# Autodesk Inventor assembly: robot_driver_board
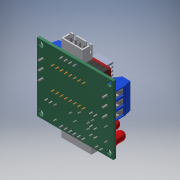
[picture p0: Inventor's stored thumbnail of the model, 180x180]
Saved by Autodesk Inventor 2019 (Build 230136000, 136)
## iProperties
Created: 2020-01-03
Part Number: robot_driver_board
Material: Типовые
Document SubType Name: Assembly
Designer: Петров Иван
Author: Петров Иван
## Documents named in this file (12)
- E:\IVAN\Ivan_desktop\GitHub\Arm_manip\electronic\3d_visualization\robot_driver_board\robot_driver_board.iam
- E:\IVAN\Ivan_desktop\GitHub\Arm_manip\electronic\3d_visualization\lib\tb5p-3p_p5_l15_w7-6_h10.ipt
- E:\IVAN\Ivan_desktop\GitHub\Arm_manip\electronic\3d_visualization\robot_driver_board\board.ipt
- E:\IVAN\Ivan_desktop\GitHub\Arm_manip\electronic\3d_visualization\lib\Female Pin Header 01x01 Pitch 2.54mm Height 8.5mm\Female Pin Header 01x01 Pitch 2.54mm Height 8.5mm.iam
- E:\IVAN\Ivan_desktop\GitHub\Arm_manip\electronic\3d_visualization\lib\A4988\A4988 RED.iam
- E:\IVAN\Ivan_desktop\GitHub\Arm_manip\electronic\3d_visualization\lib\LED 3mm (Red).ipt
- E:\IVAN\Ivan_desktop\GitHub\Arm_manip\electronic\3d_visualization\lib\JST - XH - Thru (R) - 4Pin - 2.54mm.ipt
- E:\IVAN\Ivan_desktop\GitHub\Arm_manip\electronic\3d_visualization\lib\JST - XH - Thru (R) - 6Pin - 2.54mm.ipt
- E:\IVAN\Ivan_desktop\GitHub\Arm_manip\electronic\3d_visualization\lib\JST - XH - Thru (V) - 4Pin - 2.54mm.ipt
- E:\IVAN\Ivan_desktop\GitHub\Arm_manip\electronic\3d_visualization\lib\JST - XH - Thru (V) - 6Pin - 2.54mm.ipt
- E:\IVAN\Ivan_desktop\GitHub\Arm_manip\electronic\3d_visualization\lib\1,2 kOhm R Axial DIN0207 L6.3mm D2.5mm P10.16mm Horizontal.ipt
- E:\IVAN\Ivan_desktop\GitHub\Arm_manip\electronic\3d_visualization\lib\1,0 kOhm R Axial DIN0207 L6.3mm D2.5mm P7.62mm Horizontal.ipt
## Components (34 placed, 11 different names)
1. tb5p-3p_p5_l15_w7-6_h10:1 — Совмещение:1, Совмещение:2, Совмещение:3
2. tb5p-3p_p5_l15_w7-6_h10:2 — Совмещение:4, Совмещение:5, Совмещение:6
3. board:1 — Совмещение:1, Совмещение:2, Совмещение:3, Совмещение:4, Совмещение:5, Совмещение:6, Совмещение:7, Совмещение:8, Угол:1, Совмещение:9, Совмещение:10, Угол:2, Совмещение:14, Совмещение:15, Совмещение:16, Совмещение:17, Совмещение:18, Совмещение:19, Совмещение:20, Совмещение:21, Совмещение:22, Совмещение:23, Совмещение:24, Совмещение:25, Совмещение:26, Совмещение:27, Совмещение:28, Совмещение:29, Совмещение:30, Совмещение:31, Совмещение:32, Совмещение:33, Совмещение:34, Совмещение:35, Совмещение:36, Совмещение:37, Совмещение:38, Совмещение:39, Совмещение:40, Совмещение:41, Совмещение:42, Касательность:1, Совмещение:43, Совмещение:44, Касательность:2, Касательность:3, Совмещение:45, Совмещение:46, Совмещение:47, Совмещение:48, Касательность:4, Совмещение:49, Совмещение:50, Касательность:5
4. A4988 RED:1 [sub-assembly] — Совмещение:11, Совмещение:12, Совмещение:13
5. LED 3mm (Red):1 — Совмещение:17, Совмещение:18, Совмещение:19
6. LED 3mm (Red):2 — Совмещение:14, Совмещение:15, Совмещение:16
7. LED 3mm (Red):3 — Совмещение:20, Совмещение:21, Совмещение:22
8. LED 3mm (Red):4 — Совмещение:23, Совмещение:24, Совмещение:25
9. LED 3mm (Red):5 — Совмещение:26, Совмещение:27, Совмещение:28
10. JST - XH - Thru (R) - 4Pin - 2.54mm:1 — Совмещение:29, Совмещение:30, Совмещение:31
11. JST - XH - Thru (R) - 6Pin - 2.54mm:1 — Совмещение:32, Совмещение:33, Совмещение:34
12. JST - XH - Thru (V) - 4Pin - 2.54mm:1 — Совмещение:35, Совмещение:36, Совмещение:37
13. JST - XH - Thru (V) - 6Pin - 2.54mm:1 — Совмещение:38, Совмещение:39, Совмещение:40
14. 1,2 kOhm R Axial DIN0207 L6.3mm D2.5mm P10.16mm Horizontal:1 — Совмещение:41, Совмещение:42, Касательность:1
15. 1,0 kOhm R Axial DIN0207 L6.3mm D2.5mm P7.62mm Horizontal:1 — Совмещение:43, Совмещение:44, Касательность:2
16. 1,0 kOhm R Axial DIN0207 L6.3mm D2.5mm P7.62mm Horizontal:2 — Касательность:3, Совмещение:45, Совмещение:46
17. 1,0 kOhm R Axial DIN0207 L6.3mm D2.5mm P7.62mm Horizontal:3 — Совмещение:47, Совмещение:48, Касательность:4
18. 1,0 kOhm R Axial DIN0207 L6.3mm D2.5mm P7.62mm Horizontal:4 — Совмещение:49, Совмещение:50, Касательность:5
19. Female Pin Header 01x01 Pitch 2.54mm Height 8.5mm:2 [sub-assembly] — Совмещение:9, Совмещение:10, Угол:2
20. Female Pin Header 01x01 Pitch 2.54mm Height 8.5mm:1 [sub-assembly] — Совмещение:7, Совмещение:8, Угол:1
21. Female Pin Header 01x01 Pitch 2.54mm Height 8.5mm:3 [sub-assembly]
22. Female Pin Header 01x01 Pitch 2.54mm Height 8.5mm:4 [sub-assembly]
23. Female Pin Header 01x01 Pitch 2.54mm Height 8.5mm:5 [sub-assembly]
24. Female Pin Header 01x01 Pitch 2.54mm Height 8.5mm:6 [sub-assembly]
25. Female Pin Header 01x01 Pitch 2.54mm Height 8.5mm:7 [sub-assembly]
26. Female Pin Header 01x01 Pitch 2.54mm Height 8.5mm:8 [sub-assembly]
27. Female Pin Header 01x01 Pitch 2.54mm Height 8.5mm:9 [sub-assembly]
28. Female Pin Header 01x01 Pitch 2.54mm Height 8.5mm:10 [sub-assembly]
29. Female Pin Header 01x01 Pitch 2.54mm Height 8.5mm:11 [sub-assembly]
30. Female Pin Header 01x01 Pitch 2.54mm Height 8.5mm:12 [sub-assembly]
31. Female Pin Header 01x01 Pitch 2.54mm Height 8.5mm:13 [sub-assembly]
32. Female Pin Header 01x01 Pitch 2.54mm Height 8.5mm:14 [sub-assembly] — Совмещение:11
33. Female Pin Header 01x01 Pitch 2.54mm Height 8.5mm:15 [sub-assembly] — Совмещение:12, Совмещение:13
34. Female Pin Header 01x01 Pitch 2.54mm Height 8.5mm:16 [sub-assembly]
## Component patterns: (8 elements, first: Female Pin Header 01x01 Pitch 2.54mm Height 8.5mm:2 + Female Pin Header 01x01 Pitch 2.54mm Height 8.5mm:1)
## Relationships (57: Mate 50, Tangent 5, Angle 2)
- Совмещение:1 [Mate]: tb5p-3p_p5_l15_w7-6_h10:1 ↔ board:1
- Совмещение:2 [Mate]: tb5p-3p_p5_l15_w7-6_h10:1 ↔ board:1
- Совмещение:3 [Mate]: tb5p-3p_p5_l15_w7-6_h10:1 ↔ board:1
- Совмещение:4 [Mate]: tb5p-3p_p5_l15_w7-6_h10:2 ↔ board:1
- Совмещение:5 [Mate]: tb5p-3p_p5_l15_w7-6_h10:2 ↔ board:1
- Совмещение:6 [Mate]: tb5p-3p_p5_l15_w7-6_h10:2 ↔ board:1
- Совмещение:7 [Mate]: board:1 ↔ Female Pin Header 01x01 Pitch 2.54mm Height 8.5mm:1
- Совмещение:8 [Mate]: board:1 ↔ Female Pin Header 01x01 Pitch 2.54mm Height 8.5mm:1
- Угол:1 [Angle] (0 deg): board:1 ↔ Female Pin Header 01x01 Pitch 2.54mm Height 8.5mm:1
- Совмещение:9 [Mate]: board:1 ↔ Female Pin Header 01x01 Pitch 2.54mm Height 8.5mm:2
- Совмещение:10 [Mate]: board:1 ↔ Female Pin Header 01x01 Pitch 2.54mm Height 8.5mm:2
- Угол:2 [Angle] (0 deg): board:1 ↔ Female Pin Header 01x01 Pitch 2.54mm Height 8.5mm:2
- Совмещение:11 [Mate]: A4988 RED:1 ↔ Female Pin Header 01x01 Pitch 2.54mm Height 8.5mm:14
- Совмещение:12 [Mate]: A4988 RED:1 ↔ Female Pin Header 01x01 Pitch 2.54mm Height 8.5mm:15
- Совмещение:13 [Mate]: A4988 RED:1 ↔ Female Pin Header 01x01 Pitch 2.54mm Height 8.5mm:15
- Совмещение:14 [Mate] (5 mm): board:1 ↔ LED 3mm (Red):2
- Совмещение:15 [Mate]: board:1 ↔ LED 3mm (Red):2
- Совмещение:16 [Mate]: board:1 ↔ LED 3mm (Red):2
- Совмещение:17 [Mate]: board:1 ↔ LED 3mm (Red):1
- Совмещение:18 [Mate]: board:1 ↔ LED 3mm (Red):1
- Совмещение:19 [Mate] (5 mm): board:1 ↔ LED 3mm (Red):1
- Совмещение:20 [Mate]: board:1 ↔ LED 3mm (Red):3
- Совмещение:21 [Mate]: board:1 ↔ LED 3mm (Red):3
- Совмещение:22 [Mate] (5 mm): board:1 ↔ LED 3mm (Red):3
- Совмещение:23 [Mate]: board:1 ↔ LED 3mm (Red):4
- Совмещение:24 [Mate]: board:1 ↔ LED 3mm (Red):4
- Совмещение:25 [Mate] (5 mm): board:1 ↔ LED 3mm (Red):4
- Совмещение:26 [Mate]: board:1 ↔ LED 3mm (Red):5
- Совмещение:27 [Mate]: board:1 ↔ LED 3mm (Red):5
- Совмещение:28 [Mate] (5 mm): board:1 ↔ LED 3mm (Red):5
- Совмещение:29 [Mate]: board:1 ↔ JST - XH - Thru (R) - 4Pin - 2.54mm:1
- Совмещение:30 [Mate]: board:1 ↔ JST - XH - Thru (R) - 4Pin - 2.54mm:1
- Совмещение:31 [Mate]: board:1 ↔ JST - XH - Thru (R) - 4Pin - 2.54mm:1
- Совмещение:32 [Mate]: board:1 ↔ JST - XH - Thru (R) - 6Pin - 2.54mm:1
- Совмещение:33 [Mate]: board:1 ↔ JST - XH - Thru (R) - 6Pin - 2.54mm:1
- Совмещение:34 [Mate]: board:1 ↔ JST - XH - Thru (R) - 6Pin - 2.54mm:1
- Совмещение:35 [Mate]: board:1 ↔ JST - XH - Thru (V) - 4Pin - 2.54mm:1
- Совмещение:36 [Mate]: board:1 ↔ JST - XH - Thru (V) - 4Pin - 2.54mm:1
- Совмещение:37 [Mate]: board:1 ↔ JST - XH - Thru (V) - 4Pin - 2.54mm:1
- Совмещение:38 [Mate]: board:1 ↔ JST - XH - Thru (V) - 6Pin - 2.54mm:1
- Совмещение:39 [Mate]: board:1 ↔ JST - XH - Thru (V) - 6Pin - 2.54mm:1
- Совмещение:40 [Mate]: board:1 ↔ JST - XH - Thru (V) - 6Pin - 2.54mm:1
- Совмещение:41 [Mate]: board:1 ↔ 1,2 kOhm R Axial DIN0207 L6.3mm D2.5mm P10.16mm Horizontal:1
- Совмещение:42 [Mate]: board:1 ↔ 1,2 kOhm R Axial DIN0207 L6.3mm D2.5mm P10.16mm Horizontal:1
- Касательность:1 [Tangent]: board:1 ↔ 1,2 kOhm R Axial DIN0207 L6.3mm D2.5mm P10.16mm Horizontal:1
- Совмещение:43 [Mate]: board:1 ↔ 1,0 kOhm R Axial DIN0207 L6.3mm D2.5mm P7.62mm Horizontal:1
- Совмещение:44 [Mate]: board:1 ↔ 1,0 kOhm R Axial DIN0207 L6.3mm D2.5mm P7.62mm Horizontal:1
- Касательность:2 [Tangent]: board:1 ↔ 1,0 kOhm R Axial DIN0207 L6.3mm D2.5mm P7.62mm Horizontal:1
- Касательность:3 [Tangent]: board:1 ↔ 1,0 kOhm R Axial DIN0207 L6.3mm D2.5mm P7.62mm Horizontal:2
- Совмещение:45 [Mate]: board:1 ↔ 1,0 kOhm R Axial DIN0207 L6.3mm D2.5mm P7.62mm Horizontal:2
- Совмещение:46 [Mate]: board:1 ↔ 1,0 kOhm R Axial DIN0207 L6.3mm D2.5mm P7.62mm Horizontal:2
- Совмещение:47 [Mate]: board:1 ↔ 1,0 kOhm R Axial DIN0207 L6.3mm D2.5mm P7.62mm Horizontal:3
- Совмещение:48 [Mate]: board:1 ↔ 1,0 kOhm R Axial DIN0207 L6.3mm D2.5mm P7.62mm Horizontal:3
- Касательность:4 [Tangent]: board:1 ↔ 1,0 kOhm R Axial DIN0207 L6.3mm D2.5mm P7.62mm Horizontal:3
- Совмещение:49 [Mate]: board:1 ↔ 1,0 kOhm R Axial DIN0207 L6.3mm D2.5mm P7.62mm Horizontal:4
- Совмещение:50 [Mate]: board:1 ↔ 1,0 kOhm R Axial DIN0207 L6.3mm D2.5mm P7.62mm Horizontal:4
- Касательность:5 [Tangent]: board:1 ↔ 1,0 kOhm R Axial DIN0207 L6.3mm D2.5mm P7.62mm Horizontal:4
